# Autodesk Inventor assembly: Unicycle
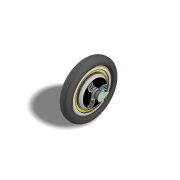
[picture p0: Inventor's stored thumbnail of the model, 180x180]
Saved by Autodesk Inventor 2020 (Build 240168000, 168)
## iProperties
Created: 2019-05-20
Part Number: Unicycle
Document SubType Name: Assembly
Designer: chitl
Author: chitl
## Documents named in this file (5)
- C:\Users\chitl\Desktop\OneWheel\Wheel Assembled\Wheel\Wheel.iam
- C:\Users\chitl\Desktop\OneWheel\Wheel Assembled\Wheel\Axle.ipt
- C:\Users\chitl\Desktop\OneWheel\Wheel Assembled\Wheel\Hub.ipt
- C:\Users\chitl\Desktop\OneWheel\Wheel Assembled\Wheel\Design.ipt
- C:\Users\chitl\Desktop\OneWheel\Wheel Assembled\Wheel\Tyre.ipt
## Components (9 placed, 4 different names)
1. Axle:1 — Rotational:1
2. Hub:1 — Rotational:1, Rigid:1, Rigid:2, Rigid:3
3. Tyre:1 — Rigid:2
4. Design:3 — Rigid:1
5. Design:4
6. Design:5
7. Design:6 — Rigid:3
8. Design:7
9. Design:8
## Component patterns: (3 elements, first: Design:3), (3 elements, first: Design:6)
## Relationships (4: WeldJoint 3, RevoluteJoint 1)
- Rotational:1 [RevoluteJoint]: Axle:1 ↔ Hub:1
- Rigid:1 [WeldJoint]: Hub:1 ↔ Design:3
- Rigid:2 [WeldJoint]: Hub:1 ↔ Tyre:1
- Rigid:3 [WeldJoint]: Hub:1 ↔ Design:6
